# Autodesk Inventor assembly: Assembly_v3.0018
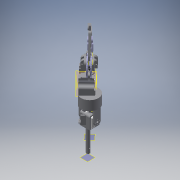
[picture p0: Inventor's stored thumbnail of the model, 180x180]
Saved by Autodesk Inventor 2018 (Build 220112000, 112)
## iProperties
Created: 2018-02-18
Part Number: Assembly_v3.0018
Document SubType Name: Assembly
Designer: Bardo91
Author: Bardo91
## Documents named in this file (17)
- C:\Users\vigus\Documents\gihug\hecatonquiros\cad_models\tools\gripper\serial_model_bearing_6DoF\Assembly_v3.0018.iam
- C:\Users\vigus\Documents\gihug\hecatonquiros\cad_models\tools\gripper\serial_model_bearing_6DoF\attachment_arm2_grande_microsevometalico.ipt
- C:\Users\vigus\Documents\gihug\hecatonquiros\cad_models\tools\gripper\serial_model_bearing_6DoF\microservo_FT_2322.ipt
- C:\Users\vigus\Documents\gihug\hecatonquiros\cad_models\tools\gripper\serial_model_bearing_6DoF\middle_joint_microservo_metalico_v2.ipt
- C:\Users\vigus\Documents\gihug\hecatonquiros\cad_models\tools\gripper\serial_model_bearing_6DoF\base_gripper_v2.ipt
- E:\programming\hecatonquiros\cad_models\accesories\gripper\barra_triangulo.ipt
- E:\programming\hecatonquiros\cad_models\accesories\gripper\barragarra_pilar_3.ipt
- C:\Users\vigus\Documents\gihug\hecatonquiros\cad_models\tools\gripper\serial_model_bearing_6DoF\ScrewActuatorGripper.ipt
- C:\Users\vigus\Documents\gihug\hecatonquiros\cad_models\tools\gripper\serial_model_bearing_6DoF\ScrewActuatorGripperCenter.ipt
- E:\programming\hecatonquiros\cad_models\accesories\gripper\garra_pilar.ipt
- C:\Users\vigus\Documents\gihug\hecatonquiros\cad_models\tools\gripper\serial_model_bearing_6DoF\microservo_FT.ipt
- C:\Users\vigus\Documents\gihug\hecatonquiros\cad_models\tools\gripper\serial_model_bearing_6DoF\bearing_19.ipt
- C:\Users\vigus\Documents\gihug\hecatonquiros\cad_models\tools\gripper\serial_model_bearing_6DoF\bearing_24.ipt
- C:\Users\vigus\Documents\gihug\hecatonquiros\cad_models\tools\gripper\serial_model_0dof\gripper.ipt
- C:\Users\vigus\Documents\gihug\hecatonquiros\cad_models\accesories\gripper\barragarra_pilar_3.ipt
- C:\Users\vigus\Documents\gihug\hecatonquiros\cad_models\accesories\gripper\barra_triangulo.ipt
- C:\Users\vigus\Documents\gihug\hecatonquiros\cad_models\accesories\gripper\garra_pilar.ipt
## Components (32 placed, 13 different names)
1. attachment_arm2_grande_microsevometalico:1 — Mate:1, Mate:3, Mate:4, Mate:5, Mate:6
2. microservo_FT_2322:1 — Mate:1, Mate:3, Mate:4
3. middle_joint_microservo_metalico_v2:1 — Mate:5, Mate:6, Mate:7, Mate:66, Mate:67, Mate:69
4. base_gripper_v2:1 — Mate:7, Mate:9, Mate:11, Mate:12, Mate:13, Mate:14, Mate:15, Mate:16, Mate:25, Mate:26, Mate:27, Mate:28, Mate:47, Mate:48, Mate:50, Mate:52, Mate:53, Mate:54, Mate:57, Mate:58, Mate:61, Mate:62, Mate:63, Mate:64, Mate:70, Mate:71, Mate:72, Mate:73, Mate:74, Mate:75, Mate:76, Mate:77, Mate:78, Mate:79, Mate:88, Mate:89, Mate:90, Mate:91, Mate:92, Mate:93, Mate:94, Mate:95
5. microservo_FT_2322:2 — Mate:9, Mate:11, Mate:12, Mate:43, Mate:68
6. barra_triangulo:1 — Mate:46, Mate:51, Mate:56, Mate:60
7. barra_triangulo:2 — Mate:45, Mate:49, Mate:55, Mate:59
8. barragarra_pilar_3:1 — Mate:13, Mate:14
9. barragarra_pilar_3:2 — Mate:15, Mate:16
10. barragarra_pilar_3:3 — Mate:25, Mate:28
11. barragarra_pilar_3:4 — Mate:26, Mate:27
12. ScrewActuatorGripper:1 — Mate:43, Mate:44, Mate:68
13. ScrewActuatorGripperCenter:1 — Mate:44, Mate:45, Mate:46, Mate:59, Mate:60, Mate:83, Mate:99
14. garra_pilar:1 — Mate:47, Mate:48, Mate:49
15. garra_pilar:2 — Mate:50, Mate:51, Mate:52
16. garra_pilar:3 — Mate:53, Mate:55, Mate:58
17. garra_pilar:4 — Mate:54, Mate:56, Mate:57
18. microservo_FT:1 — Mate:61, Mate:62, Mate:63
19. bearing_19:1 — Mate:64, Mate:69, Mate:70
20. bearing_24:1 — Mate:66, Mate:67, Mate:71
21. gripper:1 — Mate:84, Mate:85, Mate:86, Mate:87
22. gripper:2 — Mate:100, Mate:101, Mate:102, Mate:103
23. barragarra_pilar_3:5 — Mate:94, Mate:95, Mate:103
24. barragarra_pilar_3:6 — Mate:92, Mate:93, Mate:102
25. barragarra_pilar_3:7 — Mate:76, Mate:77, Mate:86
26. barragarra_pilar_3:8 — Mate:78, Mate:79, Mate:87
27. barra_triangulo:3 — Mate:80, Mate:81, Mate:82, Mate:83, Mate:84, Mate:85
28. barra_triangulo:4 — Mate:96, Mate:97, Mate:98, Mate:99, Mate:100, Mate:101
29. garra_pilar:5 — Mate:72, Mate:73, Mate:80
30. garra_pilar:6 — Mate:74, Mate:75, Mate:81, Mate:82
31. garra_pilar:7 — Mate:90, Mate:91, Mate:96, Mate:98
32. garra_pilar:8 — Mate:88, Mate:89, Mate:97
## Relationships (77: Mate 77)
- Mate:1: attachment_arm2_grande_microsevometalico:1 ↔ microservo_FT_2322:1
- Mate:3: attachment_arm2_grande_microsevometalico:1 ↔ microservo_FT_2322:1
- Mate:4: attachment_arm2_grande_microsevometalico:1 ↔ microservo_FT_2322:1
- Mate:5: attachment_arm2_grande_microsevometalico:1 ↔ middle_joint_microservo_metalico_v2:1
- Mate:6: attachment_arm2_grande_microsevometalico:1 ↔ middle_joint_microservo_metalico_v2:1
- Mate:7: middle_joint_microservo_metalico_v2:1 ↔ base_gripper_v2:1
- Mate:9: base_gripper_v2:1 ↔ microservo_FT_2322:2
- Mate:11: base_gripper_v2:1 ↔ microservo_FT_2322:2
- Mate:12: base_gripper_v2:1 ↔ microservo_FT_2322:2
- Mate:13: base_gripper_v2:1 ↔ barragarra_pilar_3:1
- Mate:14: base_gripper_v2:1 ↔ barragarra_pilar_3:1
- Mate:15: base_gripper_v2:1 ↔ barragarra_pilar_3:2
- Mate:16: base_gripper_v2:1 ↔ barragarra_pilar_3:2
- Mate:25: base_gripper_v2:1 ↔ barragarra_pilar_3:3
- Mate:26: base_gripper_v2:1 ↔ barragarra_pilar_3:4
- Mate:27: base_gripper_v2:1 ↔ barragarra_pilar_3:4
- Mate:28: base_gripper_v2:1 ↔ barragarra_pilar_3:3
- Mate:43: microservo_FT_2322:2 ↔ ScrewActuatorGripper:1
- Mate:44: ScrewActuatorGripper:1 ↔ ScrewActuatorGripperCenter:1
- Mate:45: barra_triangulo:2 ↔ ScrewActuatorGripperCenter:1
- Mate:46: barra_triangulo:1 ↔ ScrewActuatorGripperCenter:1
- Mate:47: base_gripper_v2:1 ↔ garra_pilar:1
- Mate:48: base_gripper_v2:1 ↔ garra_pilar:1
- Mate:49: barra_triangulo:2 ↔ garra_pilar:1
- Mate:50: base_gripper_v2:1 ↔ garra_pilar:2
- Mate:51: barra_triangulo:1 ↔ garra_pilar:2
- Mate:52: base_gripper_v2:1 ↔ garra_pilar:2
- Mate:53: base_gripper_v2:1 ↔ garra_pilar:3
- Mate:54: base_gripper_v2:1 ↔ garra_pilar:4
- Mate:55: barra_triangulo:2 ↔ garra_pilar:3
- Mate:56: barra_triangulo:1 ↔ garra_pilar:4
- Mate:57: base_gripper_v2:1 ↔ garra_pilar:4
- Mate:58: base_gripper_v2:1 ↔ garra_pilar:3
- Mate:59: barra_triangulo:2 ↔ ScrewActuatorGripperCenter:1
- Mate:60: barra_triangulo:1 ↔ ScrewActuatorGripperCenter:1
- Mate:61: base_gripper_v2:1 ↔ microservo_FT:1
- Mate:62: base_gripper_v2:1 ↔ microservo_FT:1
- Mate:63: base_gripper_v2:1 ↔ microservo_FT:1
- Mate:64: base_gripper_v2:1 ↔ bearing_19:1
- Mate:66: middle_joint_microservo_metalico_v2:1 ↔ bearing_24:1
- Mate:67: middle_joint_microservo_metalico_v2:1 ↔ bearing_24:1
- Mate:68: microservo_FT_2322:2 ↔ ScrewActuatorGripper:1
- Mate:69: middle_joint_microservo_metalico_v2:1 ↔ bearing_19:1
- Mate:70: base_gripper_v2:1 ↔ bearing_19:1
- Mate:71: base_gripper_v2:1 ↔ bearing_24:1
- Mate:72: base_gripper_v2:1 ↔ garra_pilar:5
- Mate:73: base_gripper_v2:1 ↔ garra_pilar:5
- Mate:74: base_gripper_v2:1 ↔ garra_pilar:6
- Mate:75: base_gripper_v2:1 ↔ garra_pilar:6
- Mate:76: base_gripper_v2:1 ↔ barragarra_pilar_3:7
- Mate:77: base_gripper_v2:1 ↔ barragarra_pilar_3:7
- Mate:78: base_gripper_v2:1 ↔ barragarra_pilar_3:8
- Mate:79: base_gripper_v2:1 ↔ barragarra_pilar_3:8
- Mate:80: barra_triangulo:3 ↔ garra_pilar:5
- Mate:81: barra_triangulo:3 ↔ garra_pilar:6
- Mate:82: barra_triangulo:3 ↔ garra_pilar:6
- Mate:83: ScrewActuatorGripperCenter:1 ↔ barra_triangulo:3
- Mate:84: gripper:1 ↔ barra_triangulo:3
- Mate:85: gripper:1 ↔ barra_triangulo:3
- Mate:86: gripper:1 ↔ barragarra_pilar_3:7
- Mate:87: gripper:1 ↔ barragarra_pilar_3:8
- Mate:88: base_gripper_v2:1 ↔ garra_pilar:8
- Mate:89: base_gripper_v2:1 ↔ garra_pilar:8
- Mate:90: base_gripper_v2:1 ↔ garra_pilar:7
- Mate:91: base_gripper_v2:1 ↔ garra_pilar:7
- Mate:92: base_gripper_v2:1 ↔ barragarra_pilar_3:6
- Mate:93: base_gripper_v2:1 ↔ barragarra_pilar_3:6
- Mate:94: base_gripper_v2:1 ↔ barragarra_pilar_3:5
- Mate:95: base_gripper_v2:1 ↔ barragarra_pilar_3:5
- Mate:96: barra_triangulo:4 ↔ garra_pilar:7
- Mate:97: barra_triangulo:4 ↔ garra_pilar:8
- Mate:98: barra_triangulo:4 ↔ garra_pilar:7
- Mate:99: ScrewActuatorGripperCenter:1 ↔ barra_triangulo:4
- Mate:100: gripper:2 ↔ barra_triangulo:4
- Mate:101: gripper:2 ↔ barra_triangulo:4
- Mate:102: gripper:2 ↔ barragarra_pilar_3:6
- Mate:103: gripper:2 ↔ barragarra_pilar_3:5
